# Autodesk Inventor assembly: Ensamble
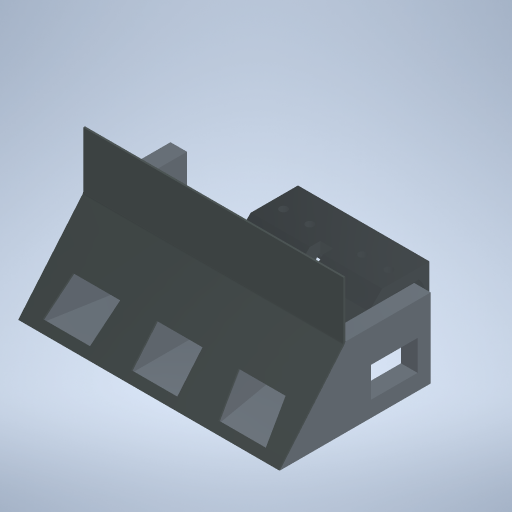
[picture p0: Inventor's stored thumbnail of the model, 512x512]
Saved by Autodesk Inventor 2024.1 (Build 281209000, 209)
## iProperties
Created: 2024-08-08
Part Number: Ensamble
Document SubType Name: Assembly
Designer: Usuario
Author: Usuario
## Documents named in this file (5)
- D:\Documentos\GitHub\Minisumo-Basic\3D Model Files\Ensamble.iam
- D:\Documentos\GitHub\Minisumo-Basic\3D Model Files\BaseTotal.ipt
- D:\Documentos\GitHub\Minisumo-Basic\3D Model Files\CajadeMotores Novamax H.ipt
- D:\Documentos\GitHub\Minisumo-Basic\3D Model Files\Cara.ipt
- D:\Documentos\GitHub\Minisumo-Basic\3D Model Files\Cuerpo.ipt
## Components (4 placed, 4 different names)
1. BaseTotal:1 — Mate:1, Flush:1, Flush:2, Mate:2, Flush:4, Flush:5, Mate:4
2. CajadeMotores Novamax H:1 — Mate:2, Flush:4, Flush:5
3. Cara:1 — Mate:3, Mate:4, Flush:6
4. Cuerpo:1 — Mate:1, Flush:1, Flush:2, Mate:3, Flush:6
## Relationships (9: Flush 5, Mate 4)
- Mate:1: BaseTotal:1 ↔ Cuerpo:1
- Flush:1: BaseTotal:1 ↔ Cuerpo:1
- Flush:2: BaseTotal:1 ↔ Cuerpo:1
- Mate:2: BaseTotal:1 ↔ CajadeMotores Novamax H:1
- Flush:4: BaseTotal:1 ↔ CajadeMotores Novamax H:1
- Flush:5: BaseTotal:1 ↔ CajadeMotores Novamax H:1
- Mate:3: Cara:1 ↔ Cuerpo:1
- Mate:4: BaseTotal:1 ↔ Cara:1
- Flush:6: Cara:1 ↔ Cuerpo:1
